# Autodesk Inventor assembly: 2in Fairlane With Hub
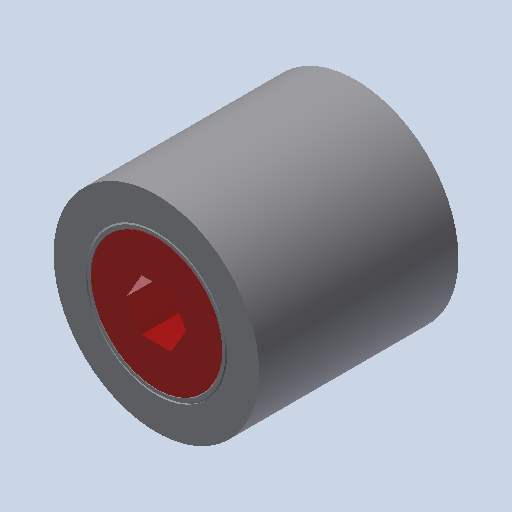
[picture p0: Inventor's stored thumbnail of the model, 512x512]
Saved by Autodesk Inventor 2023.3 (Build 273359000, 359)
## iProperties
Created: 2024-01-19
Part Number: 2in Fairlane With Hub
Document SubType Name: Assembly
Designer: slick
Author: slick
## Documents named in this file (3)
- C:\Users\mavericks\Desktop\Crescendo_2024-CAD\2024 Robot\COMMON PARTS\WHEELS\2in Fairlane With Hub.iam
- C:\Users\mavericks\Desktop\Crescendo_2024-CAD\2024 Robot\COMMON PARTS\WHEELS\2in Fairlane2476K26_Roller.ipt
- C:\Users\mavericks\Desktop\Crescendo_2024-CAD\2024 Robot\COMMON PARTS\Roller Insert.ipt
## Components (2 placed, 2 different names)
1. 2in Fairlane2476K26_Roller:1 — Mate:1, Flush:1
2. Roller Insert:1 — Mate:1, Flush:1
## Relationships (2: Mate 1, Flush 1)
- Mate:1: 2in Fairlane2476K26_Roller:1 ↔ Roller Insert:1
- Flush:1: 2in Fairlane2476K26_Roller:1 ↔ Roller Insert:1
